# Autodesk Inventor assembly: MasterAssembly
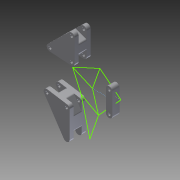
[picture p0: Inventor's stored thumbnail of the model, 180x180]
Saved by Autodesk Inventor 2011 SP2 (Build 150309200, 309)
## iProperties
Created: 2014-05-08
Part Number: MasterAssembly
Document SubType Name: Assembly
Designer: Maurice Woods
Author: Maurice Woods
## Documents named in this file (4)
- C:\Users\Maurice\Documents\GitHub\strandbeest\MasterAssembly.iam
- C:\Users\Maurice\Documents\GitHub\strandbeest\BDE.ipt
- C:\Users\Maurice\Documents\GitHub\strandbeest\GHI.ipt
- C:\Users\Maurice\Documents\Github\strandbeest\F.ipt
## Components (3 placed, 3 different names)
1. BDE:1
2. GHI:1 — Flush:1
3. F:1 — Flush:2
## Relationships (2: Flush 2)
- Flush:1: GHI:1
- Flush:2: F:1
## Named parameters: ScaleFactor = 1, LengthA = 25.4 mm, LengthB = 27.73947 mm, LengthC = 26.26896 mm, LengthD = 26.80368 mm, LengthE = 37.29789 mm, LengthF = 26.33579 mm, LengthG = 24.53104 mm, LengthH = 43.91525 mm, LengthI = 32.75254 mm, LengthJ = 33.42104 mm, LengthK = 41.37525 mm, LengthL = 5.21368 mm, LengthM = 10.02632 mm
